# Autodesk Inventor assembly: frame-back
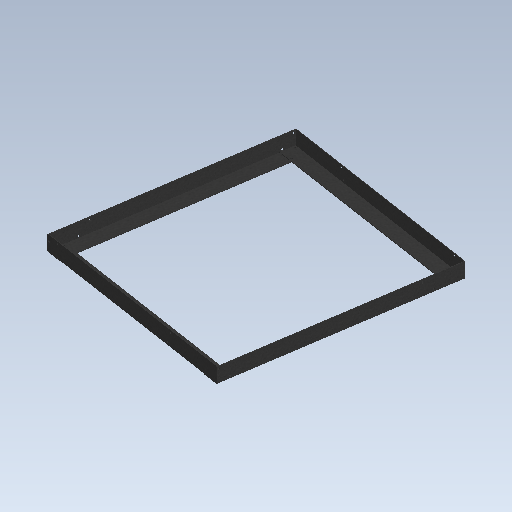
[picture p0: Inventor's stored thumbnail of the model, 512x512]
Saved by Autodesk Inventor 2020.4 (Build 244396000, 396)
## iProperties
Created: 2021-02-28
Part Number: frame-back
Document SubType Name: Assembly
Designer: AOB
Mass: 2009.86 g
Surface Area: 3311.97 cm^2
Volume: 256.033 cm^3
Density: 7.85 g/cm^3
Author: AOB
## Documents named in this file (3)
- C:\Users\marti\Documents\Inventor\ProjectBoron\Boron Ultima\frame-back.iam
- C:\Users\marti\Documents\Inventor\ProjectBoron\Boron Ultima\angleline-500.ipt
- C:\Users\marti\Documents\Inventor\ProjectBoron\Boron Ultima\angleline-400.ipt
## Components (4 placed, 2 different names)
1. angleline-500:1 — Mate:4, Mate:5, Mate:8
2. angleline-500:2 — Mate:1, Mate:6, Mate:7
3. angleline-430:1 — Mate:1, Mate:4, Mate:5
4. angleline-430:2 — Mate:6, Mate:7, Mate:8
## Relationships (6: Mate 6)
- Mate:1: angleline-500:2 ↔ angleline-430:1
- Mate:4: angleline-500:1 ↔ angleline-430:1
- Mate:5: angleline-500:1 ↔ angleline-430:1
- Mate:6: angleline-500:2 ↔ angleline-430:2
- Mate:7: angleline-500:2 ↔ angleline-430:2
- Mate:8: angleline-500:1 ↔ angleline-430:2
